# Autodesk Inventor assembly: GP5-100
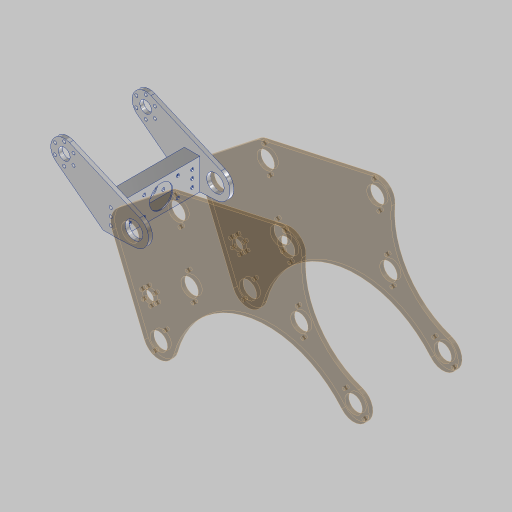
[picture p0: Inventor's stored thumbnail of the model, 512x512]
Saved by Autodesk Inventor 2023.5 (Build 275446000, 446)
## iProperties
Created: 2025-02-03
Part Number: GP5-100
Document SubType Name: Assembly
Designer: slick
Author: slick
## Documents named in this file (5)
- C:\Users\slick\OneDrive\Desktop\2025-ReefScape---CAD\Gripper\GP5\GP5-100.iam
- C:\Users\slick\OneDrive\Desktop\2025-ReefScape---CAD\Gripper\GP5\GP5-001.ipt
- C:\Users\slick\OneDrive\Desktop\2025-ReefScape---CAD\Gripper\GP5\GP5-002.ipt
- C:\Users\slick\OneDrive\Desktop\2025-ReefScape---CAD\Gripper\GP5\GP5-003.ipt
- C:\Users\slick\OneDrive\Desktop\2025-ReefScape---CAD\Gripper\GP5\GP5-004.ipt
## Components (7 placed, 4 different names)
1. GP5-001:1 — Flush:4, Mate:2, Flush:1, Flush:2, Flush:3, Flush:5
2. GP5-002:1 — Flush:4, Mate:2, Flush:5, Insert:3, Insert:4
3. GP5-002:2 — Flush:1, Flush:2, Flush:3, Insert:1, Insert:2
4. GP5-003:1 — Mate:7, Mate:9, Mate:13
5. GP5-004:1 — Insert:1, Insert:2, Mate:13
6. GP5-004:2 — Insert:3, Insert:4, Mate:11, Mate:12
7. GP5-003:2 — Mate:7, Mate:9, Mate:11, Mate:12
## Relationships (15: Mate 6, Flush 5, Insert 4)
- Flush:4: GP5-001:1 ↔ GP5-002:1
- Mate:2: GP5-001:1 ↔ GP5-002:1
- Flush:1: GP5-001:1 ↔ GP5-002:2
- Flush:2: GP5-001:1 ↔ GP5-002:2
- Flush:3: GP5-001:1 ↔ GP5-002:2
- Flush:5: GP5-001:1 ↔ GP5-002:1
- Insert:1: GP5-002:2 ↔ GP5-004:1
- Insert:2: GP5-002:2 ↔ GP5-004:1
- Insert:3: GP5-002:1 ↔ GP5-004:2
- Insert:4: GP5-002:1 ↔ GP5-004:2
- Mate:7: GP5-003:1 ↔ GP5-003:2
- Mate:9: GP5-003:1 ↔ GP5-003:2
- Mate:11: GP5-004:2 ↔ GP5-003:2
- Mate:12: GP5-004:2 ↔ GP5-003:2
- Mate:13: GP5-003:1 ↔ GP5-004:1
